# Autodesk Inventor assembly: s-assy-waight_holder
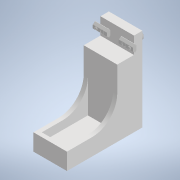
[picture p0: Inventor's stored thumbnail of the model, 180x180]
Saved by Autodesk Inventor 2022 (Build 260153000, 153)
## iProperties
Created: 2021-09-21
Part Number: s-assy-waight_holder
Document SubType Name: Assembly
Designer: yuto6
Author: yuto6
## Documents named in this file (4)
- C:\Users\yuto6\Box\Public_Share\キャチロボバトルコンテスト2021\CAD\catchrobo_hardware\assy-shooter\s-assy-waight_holder.iam
- C:\Users\yuto6\Box\Public_Share\キャチロボバトルコンテスト2021\CAD\catchrobo_hardware\assy-shooter\s_base8.ipt
- C:\Users\yuto6\Box\Public_Share\キャチロボバトルコンテスト2021\CAD\catchrobo_hardware\assy-shooter\HNTP5-5.ipt
- C:\Users\yuto6\Box\Public_Share\キャチロボバトルコンテスト2021\CAD\catchrobo_hardware\assy-shooter\CB5-15.ipt
## Components (5 placed, 3 different names)
1. s_base8:1 — メイト:1, 角度:1, 角度:2, メイト:2, メイト:3, メイト:4, メイト:5, メイト:6, メイト:7, メイト:8
2. HNTP5-5:1 — メイト:1, 角度:1, メイト:3
3. HNTP5-5:2 — 角度:2, メイト:2, メイト:4
4. CB5-15:1 — メイト:5, メイト:7
5. CB5-15:2 — メイト:6, メイト:8
## Relationships (10: Mate 8, Angle 2)
- メイト:1 [Mate]: s_base8:1 ↔ HNTP5-5:1
- 角度:1 [Angle] (0 deg): s_base8:1 ↔ HNTP5-5:1
- 角度:2 [Angle] (0 deg): s_base8:1 ↔ HNTP5-5:2
- メイト:2 [Mate]: s_base8:1 ↔ HNTP5-5:2
- メイト:3 [Mate] (1.3 mm): s_base8:1 ↔ HNTP5-5:1
- メイト:4 [Mate] (1.3 mm): s_base8:1 ↔ HNTP5-5:2
- メイト:5 [Mate]: s_base8:1 ↔ CB5-15:1
- メイト:6 [Mate]: s_base8:1 ↔ CB5-15:2
- メイト:7 [Mate]: s_base8:1 ↔ CB5-15:1
- メイト:8 [Mate]: s_base8:1 ↔ CB5-15:2
